# Autodesk Inventor assembly: FE Violet Mk V
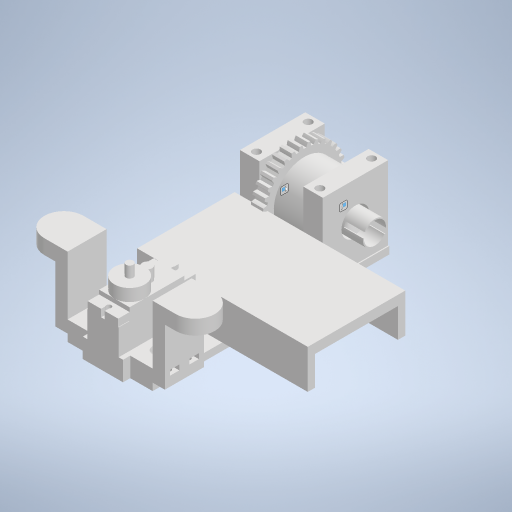
[picture p0: Inventor's stored thumbnail of the model, 512x512]
Saved by Autodesk Inventor 2023 (Build 270158000, 158)
## iProperties
Created: 2023-05-15
Part Number: FE Violet Mk V
Document SubType Name: Assembly
Designer: ivanc
Author: ivanc
## Documents named in this file (8)
- D:\Projects\Robots\FutureEngineers2023_Violet\Models\FE Violet Mk V.iam
- D:\Projects\Robots\FutureEngineers2023_Violet\Models\Enclosure components\Basis of the robot.ipt
- D:\Projects\Robots\FutureEngineers2023_Violet\Models\Electrical components\Servo SG90s.ipt
- D:\Projects\Robots\FutureEngineers2023_Violet\Models\Enclosure components\Basis of steering.ipt
- D:\Projects\Robots\FutureEngineers2023_Violet\Models\Enclosure components\Differential mount.ipt
- D:\Projects\Robots\FutureEngineers2023_Violet\Models\Mechanical components\Plastic differential with metal satellites.ipt
- D:\Projects\Robots\FutureEngineers2023_Violet\Models\Mechanical components\Bearings\Bearing 10x15x4.ipt
- D:\Projects\Robots\FutureEngineers2023_Violet\Models\Enclosure components\Battery box under the board.ipt
## Components (9 placed, 7 different names)
1. Basis of the robot:1 — Жесткий:1, Жесткий:7, Жесткий:8
2. Servo SG90s:1 — Жесткий:2
3. Basis of steering:1 — Жесткий:1, Жесткий:2
4. Differential mount:1 — Жесткий:6, Жесткий:7
5. Differential mount:2 — Жесткий:5
6. Дифференциал:1 — С поворотом:6, С поворотом:5
7. Bearing 10x15x4:1 — С поворотом:5, Жесткий:6
8. Bearing 10x15x4:2 — С поворотом:6, Жесткий:5
9. Battery box under the board:1 — Жесткий:8
## Relationships (8: WeldJoint 6, RevoluteJoint 2)
- Жесткий:1 [WeldJoint]: Basis of the robot:1 ↔ Basis of steering:1
- Жесткий:2 [WeldJoint]: Servo SG90s:1 ↔ Basis of steering:1
- С поворотом:6 [RevoluteJoint]: Дифференциал:1 ↔ Bearing 10x15x4:2
- С поворотом:5 [RevoluteJoint]: Дифференциал:1 ↔ Bearing 10x15x4:1
- Жесткий:5 [WeldJoint]: Differential mount:2 ↔ Bearing 10x15x4:2
- Жесткий:6 [WeldJoint]: Differential mount:1 ↔ Bearing 10x15x4:1
- Жесткий:7 [WeldJoint]: Basis of the robot:1 ↔ Differential mount:1
- Жесткий:8 [WeldJoint]: Basis of the robot:1 ↔ Battery box under the board:1
